# Autodesk Inventor assembly: MeinbergReceiver
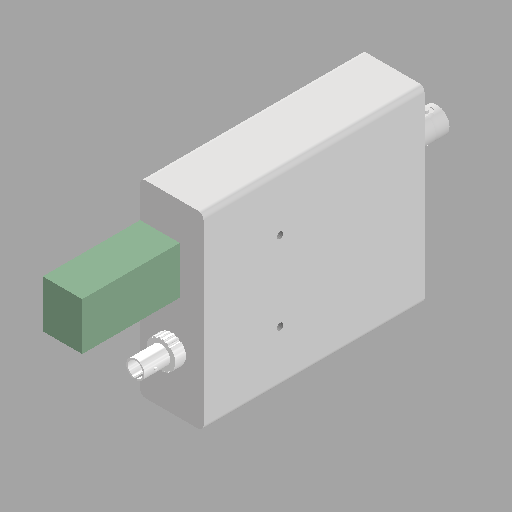
[picture p0: Inventor's stored thumbnail of the model, 512x512]
Saved by Autodesk Inventor 2025.3 (Build 293356000, 356)
## iProperties
Created: 2025-12-17
Part Number: MeinbergReceiver
Document SubType Name: Assembly
Designer: sonata
Author: sonata
## Documents named in this file (5)
- C:\Users\sonata\Documents\SetiHCRO\Front-Page\Analog-Signal-Components\RFoF\1U-Enclosure\1PPS_10MHz_RX\Parts\MeinbergReceiver.iam
- C:\Users\sonata\Documents\SetiHCRO\Front-Page\Analog-Signal-Components\RFoF\1U-Enclosure\1PPS_10MHz_RX\Parts\Meinberg_Box.ipt
- C:\Users\sonata\Documents\SetiHCRO\Front-Page\Analog-Signal-Components\RFoF\1U-Enclosure\1PPS_10MHz_RX\Parts\MeinbergPower.ipt
- D:\crush\RFoF-Meinberg\Parts\ST Bulkhead ConnectorSLDPRT\a\a.ipt
- D:\crush\RFoF-Meinberg\Parts\ST Bulkhead ConnectorSLDPRT\ST Bulkhead ConnectorSLDPRT\ST Bulkhead ConnectorSLDPRT.ipt
## Components (4 placed, 4 different names)
1. Meinberg_Box:1 — Flush:1, Mate:1, Mate:2, Flush:3, Tangent:1, Flush:4, Mate:3, Flush:5, Tangent:2
2. MeinbergPower:1 — Flush:1, Mate:1, Flush:4
3. a:1 — Mate:3, Flush:5, Tangent:2
4. ST Bulkhead ConnectorSLDPRT:1 — Mate:2, Flush:3, Tangent:1
## Relationships (9: Flush 4, Mate 3, Tangent 2)
- Flush:1 (14 mm): Meinberg_Box:1 ↔ MeinbergPower:1
- Mate:1: Meinberg_Box:1 ↔ MeinbergPower:1
- Mate:2: Meinberg_Box:1 ↔ ST Bulkhead ConnectorSLDPRT:1
- Flush:3 (8 mm): Meinberg_Box:1 ↔ ST Bulkhead ConnectorSLDPRT:1
- Tangent:1 (20 mm): Meinberg_Box:1 ↔ ST Bulkhead ConnectorSLDPRT:1
- Flush:4: Meinberg_Box:1 ↔ MeinbergPower:1
- Mate:3: Meinberg_Box:1 ↔ a:1
- Flush:5 (20 mm): Meinberg_Box:1 ↔ a:1
- Tangent:2 (10 mm): Meinberg_Box:1 ↔ a:1
